# Autodesk Inventor assembly: Assembly-jig
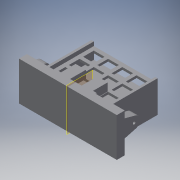
[picture p0: Inventor's stored thumbnail of the model, 180x180]
Saved by Autodesk Inventor 2018 (Build 220112000, 112)
## iProperties
Created: 2017-11-08
Part Number: Assembly-jig
Document SubType Name: Assembly
Designer: xl0
Author: xl0
## Documents named in this file (4)
- E:\Alex\koi\Cuvette-rack\Assets\renders\Assembly-jig.iam
- E:\Alex\koi\Cuvette-rack\Parts\Cuvette-rack.iam
- E:\Alex\koi\Cuvette-rack\Assets\renders\Assembly-jig-base.ipt
- C:\Users\xl0\Documents\Inventor\Content Center Files\R2018\en-US\SS-ISO 4762\ISO 4762 - M3 x 30SS-ISO.ipt
## Components (3 placed, 3 different names)
1. Cuvette-rack:1 [sub-assembly] — Flush:1, Flush:4
2. Assembly-jig-base:1 — Flush:1, Flush:4, Mate:1
3. SS ISO 4762 M3 x 30:1 — Mate:1
## Relationships (3: Flush 2, Mate 1)
- Flush:1: Cuvette-rack:1 ↔ Assembly-jig-base:1
- Flush:4 (2 mm): Cuvette-rack:1 ↔ Assembly-jig-base:1
- Mate:1: Assembly-jig-base:1 ↔ SS ISO 4762 M3 x 30:1
